# Autodesk Inventor assembly: SRF04_sur_support
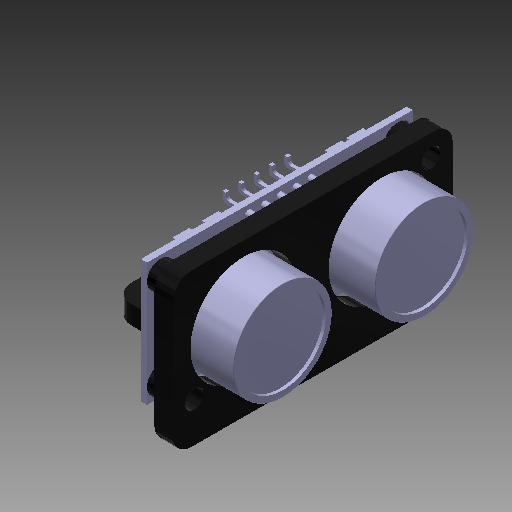
[picture p0: Inventor's stored thumbnail of the model, 512x512]
Saved by Autodesk Inventor 2019 (Build 230136000, 136)
## iProperties
Created: 2017-04-30
Part Number: SRF04_sur_support
Document SubType Name: Assembly
Designer: franc
Author: franc
## Documents named in this file (3)
- C:\Users\franc\Desktop\EsialRobotik\Mecanique\composants\SRF04\SRF04_sur_support.iam
- C:\Users\franc\Desktop\EsialRobotik\Mecanique\composants\SRF04\SRF 04.ipt
- C:\Users\franc\Desktop\EsialRobotik\Mecanique\composants\SRF04\support-srf04.ipt
## Components (2 placed, 2 different names)
1. SRF 04:1 — Mate:2, Flush:1, Mate:3
2. support-srf04:1 — Mate:2, Flush:1, Mate:3
## Relationships (3: Mate 2, Flush 1)
- Mate:2 (1 mm): SRF 04:1 ↔ support-srf04:1
- Flush:1 (1 mm): SRF 04:1 ↔ support-srf04:1
- Mate:3: SRF 04:1 ↔ support-srf04:1
